# Autodesk Inventor assembly: GGC_V1
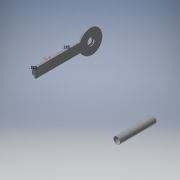
[picture p0: Inventor's stored thumbnail of the model, 180x180]
Saved by Autodesk Inventor 2016 (Build 200138000, 138)
## iProperties
Created: 2016-04-14
Part Number: GGC_V1
Document SubType Name: Assembly
Designer: rmarkowi
Author: rmarkowi
## Documents named in this file (11)
- C:\Users\rmarkowi\Documents\GGC\V1\GGC_V1.iam
- C:\Users\rmarkowi\Documents\GGC\V1\Inner Pole.ipt
- C:\Users\rmarkowi\Documents\GGC\V1\Near Gantry Bracket.ipt
- C:\Users\rmarkowi\Documents\GGC\V1\Threaded Rod.ipt
- C:\Users\rmarkowi\Documents\GGC\V1\Unthreaded Rod.ipt
- C:\Users\rmarkowi\Documents\GGC\V1\Far Gantry Bracket.ipt
- C:\Users\rmarkowi\Documents\GGC\V1\Traveller.ipt
- C:\Users\rmarkowi\Documents\GGC\V1\Threaded Rod Nut.ipt
- C:\Users\rmarkowi\Documents\GGC\V1\Threaded Rod Coupler.ipt
- C:\Users\rmarkowi\Documents\GGC\V1\NEMA23 Motor.ipt
- C:\Users\rmarkowi\Documents\GGC\V1\Arm Assembly.iam
## Components (12 placed, 10 different names)
1. Inner Pole:1
2. Threaded Rod:1 — Mate:8, Mate:9, Mate:21
3. Unthreaded Rod:1 — Mate:30, Mate:31, Mate:33
4. Unthreaded Rod:2 — Mate:6, Mate:7, Flush:1, Mate:24, Mate:32
5. Near Gantry Bracket:2 — Flush:1, Flush:2, Mate:24, Mate:25, Mate:26
6. Far Gantry Bracket:1 — Mate:6, Mate:7, Mate:8, Mate:9, Flush:2, Mate:27, Mate:28, Mate:29, Mate:30, Mate:31
7. Traveller:1 — Mate:12, Mate:13, Mate:14, Mate:15, Mate:16, Mate:17, Mate:32, Mate:33
8. Threaded Rod Nut:1 — Mate:12, Mate:13, Mate:14
9. Threaded Rod Nut:2 — Mate:15, Mate:16, Mate:17
10. Threaded Rod Coupler:1 — Mate:21, Mate:22, Mate:23
11. NEMA23 Motor:1 — Mate:22, Mate:23, Mate:25, Mate:26
12. Arm Assembly:1 [sub-assembly] — Mate:27, Mate:28, Mate:29
## Relationships (25: Mate 23, Flush 2)
- Mate:6: Unthreaded Rod:2 ↔ Far Gantry Bracket:1
- Mate:7: Unthreaded Rod:2 ↔ Far Gantry Bracket:1
- Mate:8: Threaded Rod:1 ↔ Far Gantry Bracket:1
- Mate:9: Threaded Rod:1 ↔ Far Gantry Bracket:1
- Mate:12: Traveller:1 ↔ Threaded Rod Nut:1
- Mate:13: Traveller:1 ↔ Threaded Rod Nut:1
- Mate:14: Traveller:1 ↔ Threaded Rod Nut:1
- Mate:15: Traveller:1 ↔ Threaded Rod Nut:2
- Mate:16: Traveller:1 ↔ Threaded Rod Nut:2
- Mate:17: Traveller:1 ↔ Threaded Rod Nut:2
- Mate:21: Threaded Rod:1 ↔ Threaded Rod Coupler:1
- Mate:22: Threaded Rod Coupler:1 ↔ NEMA23 Motor:1
- Mate:23: Threaded Rod Coupler:1 ↔ NEMA23 Motor:1
- Flush:1 (25.4 mm): Unthreaded Rod:2 ↔ Near Gantry Bracket:2
- Flush:2: Near Gantry Bracket:2 ↔ Far Gantry Bracket:1
- Mate:24: Unthreaded Rod:2 ↔ Near Gantry Bracket:2
- Mate:25: Near Gantry Bracket:2 ↔ NEMA23 Motor:1
- Mate:26: Near Gantry Bracket:2 ↔ NEMA23 Motor:1
- Mate:27: Far Gantry Bracket:1 ↔ Arm Assembly:1
- Mate:28: Far Gantry Bracket:1 ↔ Arm Assembly:1
- Mate:29: Far Gantry Bracket:1 ↔ Arm Assembly:1
- Mate:30: Unthreaded Rod:1 ↔ Far Gantry Bracket:1
- Mate:31: Unthreaded Rod:1 ↔ Far Gantry Bracket:1
- Mate:32: Unthreaded Rod:2 ↔ Traveller:1
- Mate:33: Unthreaded Rod:1 ↔ Traveller:1
